# Autodesk Inventor assembly: eboard1.0
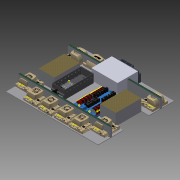
[picture p0: Inventor's stored thumbnail of the model, 180x180]
Saved by Autodesk Inventor 2014 (Build 180170000, 170)
## iProperties
Created: 2014-01-10
Part Number: eboard1.0
Document SubType Name: Assembly
Designer: pc
Author: pc
## Documents named in this file (9)
- C:\Users\robotics\Dropbox\Cad 2014 Build Season\Robot 2014\Kitbot\eboard1.0.iam
- C:\Users\robotics\Dropbox\CAD (1)\lumbrary\CAD Library v2.0\Electrical\cRIO\8-Slot cRIO.ipt
- C:\Users\robotics\Dropbox\CAD (1)\lumbrary\CAD Library v2.0\Electrical\Digital Sidecar\Digital Sidecar.iam
- C:\Users\robotics\Dropbox\CAD (1)\lumbrary\CAD Library v2.0\Electrical\Jaguar Motor Controller\Jaguar.iam
- C:\Users\robotics\Dropbox\CAD (1)\lumbrary\CAD Library v2.0\Electrical\Power Distribution Board\Power Distribution Board.iam
- C:\Users\robotics\Dropbox\CAD (1)\lumbrary\CAD Library v2.0\Electrical\Primary Circuit Breaker\Primary Circuit Breaker.iam
- C:\Users\robotics\Dropbox\CAD (1)\lumbrary\CAD Library v2.0\Electrical\Routers\Power Converter.ipt
- C:\Users\robotics\Dropbox\Cad 2014 Build Season\Robot 2014\Kitbot\eboard.ipt
- C:\Users\robotics\Dropbox\CAD (1)\lumbrary\CAD Library v2.0\Electrical\Battery\Battery.iam
## Components (16 placed, 8 different names)
1. 8-Slot cRIO:1 — Mate:12
2. Digital Sidecar:1 [sub-assembly] — Mate:11
3. Jaguar:1 [sub-assembly] — Mate:1
4. Jaguar:2 [sub-assembly] — Mate:2
5. Jaguar:3 [sub-assembly] — Mate:3
6. Jaguar:4 [sub-assembly] — Mate:4
7. Jaguar:5 [sub-assembly] — Mate:5
8. Jaguar:6 [sub-assembly] — Mate:6
9. Jaguar:7 [sub-assembly] — Mate:7
10. Jaguar:8 [sub-assembly] — Mate:8
11. Jaguar:9 [sub-assembly] — Mate:9
12. Power Distribution Board:1 [sub-assembly] — Mate:10
13. Primary Circuit Breaker:1 [sub-assembly] — Mate:13
14. Power Converter:1 — Mate:14
15. eboard:1 — Mate:1, Mate:2, Mate:3, Mate:4, Mate:5, Mate:6, Mate:7, Mate:8, Mate:9, Mate:10, Mate:11, Mate:12, Mate:13, Mate:14, Flush:1, Mate:15, Flush:2
16. Battery:1 [sub-assembly] — Flush:1, Mate:15, Flush:2
## Relationships (17: Mate 15, Flush 2)
- Mate:1: Jaguar:1 ↔ eboard:1
- Mate:2: Jaguar:2 ↔ eboard:1
- Mate:3: Jaguar:3 ↔ eboard:1
- Mate:4: Jaguar:4 ↔ eboard:1
- Mate:5: Jaguar:5 ↔ eboard:1
- Mate:6: Jaguar:6 ↔ eboard:1
- Mate:7: Jaguar:7 ↔ eboard:1
- Mate:8: Jaguar:8 ↔ eboard:1
- Mate:9: Jaguar:9 ↔ eboard:1
- Mate:10: Power Distribution Board:1 ↔ eboard:1
- Mate:11: Digital Sidecar:1 ↔ eboard:1
- Mate:12: 8-Slot cRIO:1 ↔ eboard:1
- Mate:13: Primary Circuit Breaker:1 ↔ eboard:1
- Mate:14: Power Converter:1 ↔ eboard:1
- Flush:1 (225.552 mm): eboard:1 ↔ Battery:1
- Mate:15: eboard:1 ↔ Battery:1
- Flush:2: eboard:1 ↔ Battery:1
